# Autodesk Inventor assembly: Two simple doors with glass
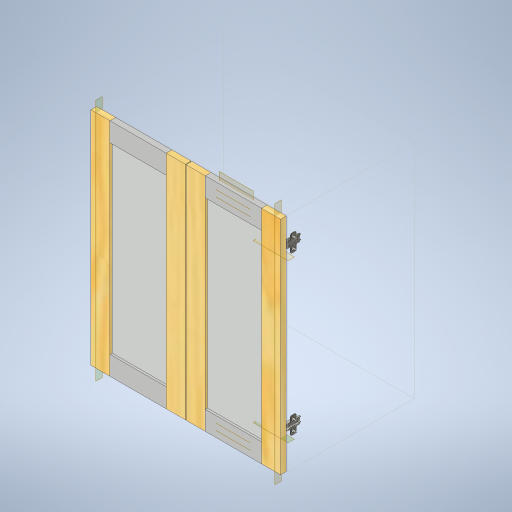
[picture p0: Inventor's stored thumbnail of the model, 512x512]
Saved by Autodesk Inventor 2024 (Build 280153000, 153)
## iProperties
RuleStatus: InUse
Created: 2017-04-13
Part Number: Two simple doors with glass
Document SubType Name: Assembly
Designer: SvetlanaB
Author: SvetlanaB
## Documents named in this file (17)
- C:\W4INV 2024 Design\iBOX LIBRARY\Kitchen\Doors\Two doors with glass\Two doors with glass.iam
- C:\W4INV 2024 Design\iBOX LIBRARY\Kitchen\Doors\Two doors with glass\Left door left panel.ipt
- C:\W4INV 2024 Design\iBOX LIBRARY\Kitchen\Doors\Two doors with glass\Left door right panel.ipt
- C:\W4INV 2024 Design\iBOX LIBRARY\Kitchen\Doors\Two doors with glass\Left door bottom panel.ipt
- C:\W4INV 2024 Design\iBOX LIBRARY\Kitchen\Doors\Two doors with glass\Left door top panel.ipt
- C:\W4INV 2024 Design\iBOX LIBRARY\Kitchen\Doors\Two doors with glass\Right door left panel.ipt
- C:\W4INV 2024 Design\iBOX LIBRARY\Kitchen\Doors\Two doors with glass\Right door right panel.ipt
- C:\W4INV 2024 Design\iBOX LIBRARY\Kitchen\Doors\Two doors with glass\Right door bottom panel.ipt
- C:\W4INV 2024 Design\iBOX LIBRARY\Kitchen\Doors\Two doors with glass\Right door top panel.ipt
- C:\W4INV 2024 Design\iBOX LIBRARY\Kitchen\Doors\Two doors with glass\Right glass.ipt
- C:\W4INV 2024 Design\iBOX LIBRARY\Kitchen\Doors\Two doors with glass\Left glass.ipt
- C:\W4INV 2024 Design\iBOX LIBRARY\Kitchen\Doors\Two doors with glass\Two simple doors with glass.ipt
- C:\W4INV 2024 Design\_LIBRARY\Hinges\CONCEALED HINGE\Full Overlay Hinge Wood Screw Cup Wood Screw T18.iam
- C:\W4INV 2024 Design\_LIBRARY\Fixed joints\Dowel\DOWEL V2\Dowel 8x30 PB T=18.ipt
- C:\W4INV 2023 Design\LIBRARY\Hinges\CONCEALED HINGE.iam
- C:\W4INV 2023 Design\LIBRARY\Fixed joints\Dowel\DOWEL V2.ipt
- C:\W4INV 2022 Design\iBOX LIBRARY\Kitchen\Doors\Two doors with glass\Two doors with glass.iam
## Components (31 placed, 13 different names)
1. @Skeleton
2. Left door left panel:1 — Flush:4, Mate:5, Mate:7, Pillar Board Plane:11, Pillar Board Plane:12, Pillar Board Plane:13, Pillar Board Plane:14
3. Left door right panel:1 — Pillar Board Plane:9, Pillar Board Plane:10, Pillar Board Plane:15, Pillar Board Plane:16
4. Left door bottom panel:1 — Nestled Board Plane:13, Nestled Board Plane:14, Nestled Board Plane:15, Nestled Board Plane:16
5. Left door top panel:1 — Nestled Board Plane:9, Nestled Board Plane:10, Nestled Board Plane:11, Nestled Board Plane:12
6. Right door left panel:1 — Pillar Board Plane:3, Pillar Board Plane:4, Pillar Board Plane:7, Pillar Board Plane:8
7. Right door right panel:1 — Flush:1, Flush:2, Flush:3, Mate:1, Mate:3, Pillar Board Plane:1, Pillar Board Plane:2, Pillar Board Plane:5, Pillar Board Plane:6
8. Right door bottom panel:1 — Flush:11, Flush:12, Nestled Board Plane:5, Nestled Board Plane:6, Nestled Board Plane:7, Nestled Board Plane:8
9. Right door top panel:1 — Flush:9, Flush:10, Flush:13, Nestled Board Plane:1, Nestled Board Plane:2, Nestled Board Plane:3, Nestled Board Plane:4
10. Right glass:1
11. Left glass:1
12. Full Overlay Hinge Wood Screw Cup Wood Screw T18:1 [sub-assembly] — Mate:1, Flush:5, Mate:2
13. Full Overlay Hinge Wood Screw Cup Wood Screw T18:2 [sub-assembly] — Mate:3, Flush:6, Mate:4
14. Full Overlay Hinge Wood Screw Cup Wood Screw T18:3 [sub-assembly] — Mate:5, Flush:7, Mate:6
15. Full Overlay Hinge Wood Screw Cup Wood Screw T18:4 [sub-assembly] — Mate:7, Flush:8, Mate:8
16. Dowel 8x30 PB T=18:1 — Axis Plane:1, Second Axis Plane:1, Nestled Board Plane:1, Pillar Board Plane:1
17. Dowel 8x30 PB T=18:2 — Nestled Board Plane:2, Axis Plane:2, Second Axis Plane:2, Pillar Board Plane:2
18. Dowel 8x30 PB T=18:3 — Nestled Board Plane:3, Axis Plane:3, Second Axis Plane:3, Pillar Board Plane:3
19. Dowel 8x30 PB T=18:4 — Nestled Board Plane:4, Axis Plane:4, Second Axis Plane:4, Pillar Board Plane:4
20. Dowel 8x30 PB T=18:5 — Nestled Board Plane:5, Axis Plane:5, Second Axis Plane:5, Pillar Board Plane:5
21. Dowel 8x30 PB T=18:6 — Nestled Board Plane:6, Axis Plane:6, Second Axis Plane:6, Pillar Board Plane:6
22. Dowel 8x30 PB T=18:7 — Nestled Board Plane:7, Axis Plane:7, Second Axis Plane:7, Pillar Board Plane:7
23. Dowel 8x30 PB T=18:8 — Nestled Board Plane:8, Axis Plane:8, Second Axis Plane:8, Pillar Board Plane:8
24. Dowel 8x30 PB T=18:9 — Nestled Board Plane:9, Axis Plane:9, Second Axis Plane:9, Pillar Board Plane:9
25. Dowel 8x30 PB T=18:10 — Nestled Board Plane:10, Axis Plane:10, Second Axis Plane:10, Pillar Board Plane:10
26. Dowel 8x30 PB T=18:11 — Nestled Board Plane:11, Axis Plane:11, Second Axis Plane:11, Pillar Board Plane:13
27. Dowel 8x30 PB T=18:12 — Nestled Board Plane:12, Axis Plane:12, Second Axis Plane:12, Pillar Board Plane:14
28. Dowel 8x30 PB T=18:13 — Nestled Board Plane:13, Axis Plane:13, Second Axis Plane:13, Pillar Board Plane:12
29. Dowel 8x30 PB T=18:14 — Nestled Board Plane:14, Axis Plane:14, Second Axis Plane:14, Pillar Board Plane:11
30. Dowel 8x30 PB T=18:15 — Nestled Board Plane:15, Axis Plane:15, Second Axis Plane:15, Pillar Board Plane:15
31. Dowel 8x30 PB T=18:16 — Nestled Board Plane:16, Axis Plane:16, Second Axis Plane:16, Pillar Board Plane:16
## Relationships (85: Mate 72, Flush 13)
- Flush:1 (-100 mm): Right door right panel:1
- Flush:2 (-100 mm): Right door right panel:1
- Flush:3 (-16.5 mm): Right door right panel:1
- Flush:4 (-16.5 mm): Left door left panel:1
- Mate:1: Right door right panel:1 ↔ Full Overlay Hinge Wood Screw Cup Wood Screw T18:1
- Flush:5: Full Overlay Hinge Wood Screw Cup Wood Screw T18:1
- Mate:2: Full Overlay Hinge Wood Screw Cup Wood Screw T18:1
- Mate:3: Right door right panel:1 ↔ Full Overlay Hinge Wood Screw Cup Wood Screw T18:2
- Flush:6: Full Overlay Hinge Wood Screw Cup Wood Screw T18:2
- Mate:4: Full Overlay Hinge Wood Screw Cup Wood Screw T18:2
- Mate:5: Left door left panel:1 ↔ Full Overlay Hinge Wood Screw Cup Wood Screw T18:3
- Flush:7: Full Overlay Hinge Wood Screw Cup Wood Screw T18:3
- Mate:6: Full Overlay Hinge Wood Screw Cup Wood Screw T18:3
- Mate:7: Left door left panel:1 ↔ Full Overlay Hinge Wood Screw Cup Wood Screw T18:4
- Flush:8: Full Overlay Hinge Wood Screw Cup Wood Screw T18:4
- Mate:8: Full Overlay Hinge Wood Screw Cup Wood Screw T18:4
- Flush:9 (-20 mm): Right door top panel:1
- Flush:10 (-20 mm): Right door top panel:1
- Flush:11 (-20 mm): Right door bottom panel:1
- Flush:12 (-20 mm): Right door bottom panel:1
- Flush:13 (-9 mm): Right door top panel:1
- Axis Plane:1 [Mate]: Dowel 8x30 PB T=18:1
- Second Axis Plane:1 [Mate]: Dowel 8x30 PB T=18:1
- Nestled Board Plane:1 [Mate]: Right door top panel:1 ↔ Dowel 8x30 PB T=18:1
- Nestled Board Plane:2 [Mate]: Right door top panel:1 ↔ Dowel 8x30 PB T=18:2
- Axis Plane:2 [Mate]: Dowel 8x30 PB T=18:2
- Second Axis Plane:2 [Mate]: Dowel 8x30 PB T=18:2
- Pillar Board Plane:1 [Mate] (-9 mm): Right door right panel:1 ↔ Dowel 8x30 PB T=18:1
- Pillar Board Plane:2 [Mate] (-9 mm): Right door right panel:1 ↔ Dowel 8x30 PB T=18:2
- Nestled Board Plane:3 [Mate]: Right door top panel:1 ↔ Dowel 8x30 PB T=18:3
- Axis Plane:3 [Mate]: Dowel 8x30 PB T=18:3
- Second Axis Plane:3 [Mate]: Dowel 8x30 PB T=18:3
- Nestled Board Plane:4 [Mate]: Right door top panel:1 ↔ Dowel 8x30 PB T=18:4
- Axis Plane:4 [Mate]: Dowel 8x30 PB T=18:4
- Second Axis Plane:4 [Mate]: Dowel 8x30 PB T=18:4
- Pillar Board Plane:3 [Mate] (-9 mm): Right door left panel:1 ↔ Dowel 8x30 PB T=18:3
- Pillar Board Plane:4 [Mate] (-9 mm): Right door left panel:1 ↔ Dowel 8x30 PB T=18:4
- Nestled Board Plane:5 [Mate]: Right door bottom panel:1 ↔ Dowel 8x30 PB T=18:5
- Axis Plane:5 [Mate]: Dowel 8x30 PB T=18:5
- Second Axis Plane:5 [Mate]: Dowel 8x30 PB T=18:5
- Nestled Board Plane:6 [Mate]: Right door bottom panel:1 ↔ Dowel 8x30 PB T=18:6
- Axis Plane:6 [Mate]: Dowel 8x30 PB T=18:6
- Second Axis Plane:6 [Mate]: Dowel 8x30 PB T=18:6
- Pillar Board Plane:5 [Mate] (-9 mm): Right door right panel:1 ↔ Dowel 8x30 PB T=18:5
- Pillar Board Plane:6 [Mate] (-9 mm): Right door right panel:1 ↔ Dowel 8x30 PB T=18:6
- Nestled Board Plane:7 [Mate]: Right door bottom panel:1 ↔ Dowel 8x30 PB T=18:7
- Axis Plane:7 [Mate]: Dowel 8x30 PB T=18:7
- Second Axis Plane:7 [Mate]: Dowel 8x30 PB T=18:7
- Nestled Board Plane:8 [Mate]: Right door bottom panel:1 ↔ Dowel 8x30 PB T=18:8
- Axis Plane:8 [Mate]: Dowel 8x30 PB T=18:8
- Second Axis Plane:8 [Mate]: Dowel 8x30 PB T=18:8
- Pillar Board Plane:7 [Mate] (-9 mm): Right door left panel:1 ↔ Dowel 8x30 PB T=18:7
- Pillar Board Plane:8 [Mate] (-9 mm): Right door left panel:1 ↔ Dowel 8x30 PB T=18:8
- Nestled Board Plane:9 [Mate]: Left door top panel:1 ↔ Dowel 8x30 PB T=18:9
- Axis Plane:9 [Mate]: Dowel 8x30 PB T=18:9
- Second Axis Plane:9 [Mate]: Dowel 8x30 PB T=18:9
- Nestled Board Plane:10 [Mate]: Left door top panel:1 ↔ Dowel 8x30 PB T=18:10
- Axis Plane:10 [Mate]: Dowel 8x30 PB T=18:10
- Second Axis Plane:10 [Mate]: Dowel 8x30 PB T=18:10
- Pillar Board Plane:9 [Mate] (-9 mm): Left door right panel:1 ↔ Dowel 8x30 PB T=18:9
- Pillar Board Plane:10 [Mate] (-9 mm): Left door right panel:1 ↔ Dowel 8x30 PB T=18:10
- Nestled Board Plane:11 [Mate]: Left door top panel:1 ↔ Dowel 8x30 PB T=18:11
- Axis Plane:11 [Mate]: Dowel 8x30 PB T=18:11
- Second Axis Plane:11 [Mate]: Dowel 8x30 PB T=18:11
- Nestled Board Plane:12 [Mate]: Left door top panel:1 ↔ Dowel 8x30 PB T=18:12
- Axis Plane:12 [Mate]: Dowel 8x30 PB T=18:12
- Second Axis Plane:12 [Mate]: Dowel 8x30 PB T=18:12
- Nestled Board Plane:13 [Mate]: Left door bottom panel:1 ↔ Dowel 8x30 PB T=18:13
- Axis Plane:13 [Mate]: Dowel 8x30 PB T=18:13
- Second Axis Plane:13 [Mate]: Dowel 8x30 PB T=18:13
- Nestled Board Plane:14 [Mate]: Left door bottom panel:1 ↔ Dowel 8x30 PB T=18:14
- Axis Plane:14 [Mate]: Dowel 8x30 PB T=18:14
- Second Axis Plane:14 [Mate]: Dowel 8x30 PB T=18:14
- Pillar Board Plane:11 [Mate] (-9 mm): Left door left panel:1 ↔ Dowel 8x30 PB T=18:14
- Pillar Board Plane:12 [Mate] (-9 mm): Left door left panel:1 ↔ Dowel 8x30 PB T=18:13
- Pillar Board Plane:13 [Mate] (-9 mm): Left door left panel:1 ↔ Dowel 8x30 PB T=18:11
- Pillar Board Plane:14 [Mate] (-9 mm): Left door left panel:1 ↔ Dowel 8x30 PB T=18:12
- Nestled Board Plane:15 [Mate]: Left door bottom panel:1 ↔ Dowel 8x30 PB T=18:15
- Axis Plane:15 [Mate]: Dowel 8x30 PB T=18:15
- Second Axis Plane:15 [Mate]: Dowel 8x30 PB T=18:15
- Nestled Board Plane:16 [Mate]: Left door bottom panel:1 ↔ Dowel 8x30 PB T=18:16
- Axis Plane:16 [Mate]: Dowel 8x30 PB T=18:16
- Second Axis Plane:16 [Mate]: Dowel 8x30 PB T=18:16
- Pillar Board Plane:15 [Mate] (-9 mm): Left door right panel:1 ↔ Dowel 8x30 PB T=18:15
- Pillar Board Plane:16 [Mate] (-9 mm): Left door right panel:1 ↔ Dowel 8x30 PB T=18:16
## Named parameters: Width = 600 mm, Depth = 400 mm, Height = 700 mm, Top_offset = 1.5 mm, Bottom_offset = 1.5 mm, Left_offset = 1.5 mm, Right_offset = 1.5 mm, Type = 1, Panel_thickness = 18 mm, Front_offset = 2 mm, Spacing_between_doors = 3 mm, Hinge_side_offset = 18 mm, Hinge_top_offset = 100 mm, Hinge_bottom_offset = 100 mm, Carcass_thickness = 60 mm
